# Autodesk Inventor assembly: camera_modul
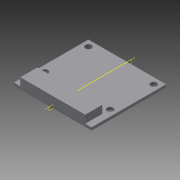
[picture p0: Inventor's stored thumbnail of the model, 180x180]
Saved by Autodesk Inventor 2014 (Build 180170000, 170)
## iProperties
Created: 2013-09-08
Part Number: camera_modul
Document SubType Name: Assembly
Designer: Felix
Author: Felix
## Documents named in this file (4)
- C:\Users\hanse\Desktop\Beep\Hardware\3D-CAD\parts\electronic\RaspberryPi_Camera\camera_modul.iam
- C:\Users\hanse\Desktop\Beep\Hardware\3D-CAD\parts\electronic\RaspberryPi_Camera\pcb.ipt
- C:\Users\hanse\Desktop\Beep\Hardware\3D-CAD\parts\electronic\RaspberryPi_Camera\connector.ipt
- C:\Users\hanse\Desktop\Beep\Hardware\3D-CAD\parts\electronic\RaspberryPi_Camera\camera.ipt
## Components (3 placed, 3 different names)
1. pcb:1 — Passend:1, Fluchtend:1, Fluchtend:2, Passend:2, Passend:3, Fluchtend:3
2. connector:1 — Passend:1, Fluchtend:1, Fluchtend:2
3. camera:1 — Passend:2, Passend:3, Fluchtend:3
## Relationships (6: Mate 3, Flush 3)
- Passend:1 [Mate]: pcb:1 ↔ connector:1
- Fluchtend:1 [Flush]: pcb:1 ↔ connector:1
- Fluchtend:2 [Flush] (2.05 mm): pcb:1 ↔ connector:1
- Passend:2 [Mate]: pcb:1 ↔ camera:1
- Passend:3 [Mate]: pcb:1 ↔ camera:1
- Fluchtend:3 [Flush] (-5.5 mm): pcb:1 ↔ camera:1
